# Autodesk Inventor assembly: SeatAssembly
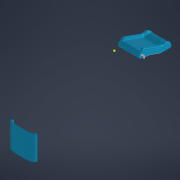
[picture p0: Inventor's stored thumbnail of the model, 180x180]
Saved by Autodesk Inventor 2021 (Build 250183000, 183)
## iProperties
Created: 2021-01-30
Part Number: SeatAssembly
Document SubType Name: Assembly
Designer: argon
Author: argon
## Documents named in this file (5)
- C:\Users\argon\OneDrive\Documents\GrabCAD\EngOne Maroons\TestSeat\SeatAssembly.iam
- C:\Users\argon\OneDrive\Documents\GrabCAD\EngOne Maroons\TestSeat\SeatBack.ipt
- C:\Users\argon\OneDrive\Documents\GrabCAD\EngOne Maroons\TestSeat\SteelPost.ipt
- C:\Users\argon\OneDrive\Documents\GrabCAD\EngOne Maroons\TestSeat\SteelBack.ipt
- C:\Users\argon\OneDrive\Documents\GrabCAD\EngOne Maroons\TestSeat\SeatBase.ipt
## Components (5 placed, 4 different names)
1. SeatBack:1 — Mate:1, Mate:2, Mate:3, Mate:4, Mate:7, Mate:8, Mate:9
2. SteelPost:1 — Mate:1, Mate:4, Mate:5
3. SteelPost:2 — Mate:2, Mate:3, Mate:5
4. SteelBack:1 — Mate:7, Mate:8, Mate:9
5. SeatBase:1
## Relationships (8: Mate 8)
- Mate:1: SeatBack:1 ↔ SteelPost:1
- Mate:2: SeatBack:1 ↔ SteelPost:2
- Mate:3: SeatBack:1 ↔ SteelPost:2
- Mate:4: SeatBack:1 ↔ SteelPost:1
- Mate:5: SteelPost:1 ↔ SteelPost:2
- Mate:7: SeatBack:1 ↔ SteelBack:1
- Mate:8: SeatBack:1 ↔ SteelBack:1
- Mate:9: SeatBack:1 ↔ SteelBack:1
